# Autodesk Inventor assembly: frame
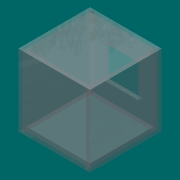
[picture p0: Inventor's stored thumbnail of the model, 180x180]
Saved by Autodesk Inventor 2016 (Build 200138000, 138)
## iProperties
Created: 2015-10-13
Part Number: frame
Document SubType Name: Assembly
Designer: Sawaiz
Author: Sawaiz
## Documents named in this file (5)
- C:\Users\Sawaiz\OneDrive\projects\modularRICH\frame\frame.iam
- C:\Users\Sawaiz\OneDrive\projects\modularRICH\frame\front.ipt
- C:\Users\Sawaiz\OneDrive\projects\modularRICH\frame\sides.ipt
- C:\Users\Sawaiz\OneDrive\projects\modularRICH\frame\topBottom.ipt
- C:\Users\Sawaiz\OneDrive\projects\modularRICH\frame\back.ipt
## Components (6 placed, 4 different names)
1. front:1 — Flush:1, Flush:2, Flush:3, Flush:4, Mate:1, Mate:2, Mate:6
2. sides:1 — Flush:1, Flush:3, Mate:2, Flush:6, Flush:7, Mate:3
3. sides:2 — Flush:2, Flush:4, Mate:1, Flush:5, Flush:8, Mate:4, Mate:7
4. topBottom:1 — Flush:5, Mate:6, Mate:7
5. topBottom:2 — Flush:6, Mate:4, Mate:5
6. back:1 — Flush:7, Mate:3, Flush:8, Mate:5
## Relationships (15: Flush 8, Mate 7)
- Flush:1: front:1 ↔ sides:1
- Flush:2: front:1 ↔ sides:2
- Flush:3: front:1 ↔ sides:1
- Flush:4: front:1 ↔ sides:2
- Mate:1: front:1 ↔ sides:2
- Mate:2: front:1 ↔ sides:1
- Flush:5: sides:2 ↔ topBottom:1
- Flush:6: sides:1 ↔ topBottom:2
- Flush:7: sides:1 ↔ back:1
- Mate:3: sides:1 ↔ back:1
- Flush:8: sides:2 ↔ back:1
- Mate:4: sides:2 ↔ topBottom:2
- Mate:5: topBottom:2 ↔ back:1
- Mate:6: front:1 ↔ topBottom:1
- Mate:7: sides:2 ↔ topBottom:1
